# Autodesk Inventor assembly: KNEE_DRIVER_ASM
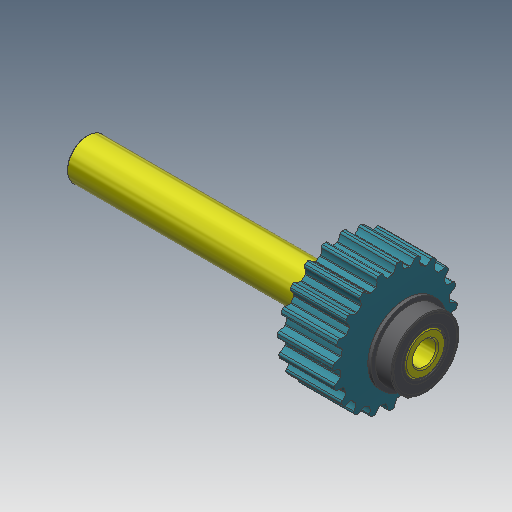
[picture p0: Inventor's stored thumbnail of the model, 512x512]
Saved by Autodesk Inventor 2019.4 (Build 234330000, 330)
## iProperties
Created: 2019-11-12
Part Number: KNEE_DRIVER_ASM
Material: 一般
Document SubType Name: Assembly
Designer: y6tada
Mass: 2.76189 g
Surface Area: 33.3674 cm^2
Volume: 2.76189 cm^3
Density: 1 g/cm^3
Author: y6tada
## Documents named in this file (4)
- C:\Workspace\Yuni9\Inventor\Asm\UPPER_LEG\KNEE_DRIVER_ASM.iam
- C:\Workspace\Yuni9\Inventor\Asm\TIMING_PULLEY\TIMING_BELT_P20.ipt
- C:\Workspace\Yuni9\Inventor\Asm\UPPER_LEG\KNEE_DRIVER_SHAFT.ipt
- C:\Workspace\Yuni9\Inventor\Libs\NSK Bearing\NSK_RB_MF106ZZ1\MF106ZZ1.iam
## Components (3 placed, 3 different names)
1. TIMING_BELT_P20:1 — メイト:3, メイト:5
2. KNEE_DRIVER_SHAFT:1 — メイト:1, メイト:2, メイト:3, メイト:4, フラッシュ:1
3. MF106ZZ1:1 [sub-assembly] — メイト:4, フラッシュ:1, メイト:5
## Relationships (6: Mate 5, Flush 1)
- メイト:1 [Mate]: KNEE_DRIVER_SHAFT:1
- メイト:2 [Mate]: KNEE_DRIVER_SHAFT:1
- メイト:3 [Mate]: TIMING_BELT_P20:1 ↔ KNEE_DRIVER_SHAFT:1
- メイト:4 [Mate]: KNEE_DRIVER_SHAFT:1 ↔ MF106ZZ1:1
- フラッシュ:1 [Flush]: KNEE_DRIVER_SHAFT:1 ↔ MF106ZZ1:1
- メイト:5 [Mate] (1.5 mm): TIMING_BELT_P20:1 ↔ MF106ZZ1:1
